# Autodesk Inventor assembly: WedgeBotV3.1
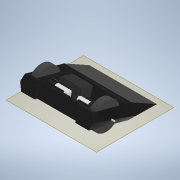
[picture p0: Inventor's stored thumbnail of the model, 180x180]
Saved by Autodesk Inventor 2020 (Build 240168000, 168)
## iProperties
Created: 2023-12-06
Part Number: WedgeBotV3.1
Document SubType Name: Assembly
Designer: smz3rm
Mass: 461.451 g
Surface Area: 1134.27 cm^2
Volume: 369.635 cm^3
Density: 1.2484 g/cm^3
Author: smz3rm
## Documents named in this file (8)
- C:\Users\smz3rm\OneDrive - BP\Documents\DigitalTwin\Models\BattleBot\WedgeBotV3.1.iam
- C:\Users\smz3rm\OneDrive - BP\Documents\DigitalTwin\Models\BattleBot\BodyWedgeWedgeV3.1.ipt
- C:\Users\smz3rm\OneDrive - BP\Documents\DigitalTwin\Models\BattleBot\BodyWedgeBaseV3.1.ipt
- C:\Users\smz3rm\OneDrive - BP\Documents\DigitalTwin\Models\BattleBot\DriveMotorV2.ipt
- C:\Users\smz3rm\OneDrive - BP\Documents\DigitalTwin\Models\BattleBot\BodyWedgeSideV3.1.ipt
- C:\Users\smz3rm\OneDrive - BP\Documents\DigitalTwin\Models\BattleBot\WheelV1.ipt
- C:\Users\smz3rm\OneDrive - BP\Documents\DigitalTwin\Models\BattleBot\HubV2.ipt
- C:\Users\smz3rm\OneDrive - BP\Documents\DigitalTwin\Models\BattleBot\BatteryV1.ipt
## Components (11 placed, 7 different names)
1. BodyWedgeWedgeV3.1:1 — Mate:1, Mate:2, Mate:3, Mate:9, Mate:12, Mate:23
2. BodyWedgeBaseV3.1:1 — Mate:1, Mate:2, Mate:3, Mate:4, Mate:5, Mate:6, Mate:7, Mate:8, Mate:10, Mate:11, Mate:13, Mate:14, Mate:20, Mate:22, Mate:24, Mate:25, Mate:26
3. DriveMotorV2:1 — Mate:7, Mate:8, Mate:19
4. DriveMotorV2:2 — Mate:4, Mate:5, Mate:6, Mate:21
5. BodyWedgeSideV3.1:1 — Mate:12, Mate:13, Mate:14
6. BodyWedgeSideV3.1:2 — Mate:9, Mate:10, Mate:11
7. WheelV1:1 — Mate:15, Mate:16
8. HubV2:1 — Mate:15, Mate:16, Mate:19, Mate:20
9. WheelV1:2 — Mate:17, Mate:18, Tangent:1
10. HubV2:2 — Mate:17, Mate:18, Mate:21, Mate:22
11. BatteryV1:1 — Mate:24, Mate:25, Mate:26
## Relationships (27: Mate 26, Tangent 1)
- Mate:1: BodyWedgeWedgeV3.1:1 ↔ BodyWedgeBaseV3.1:1
- Mate:2: BodyWedgeWedgeV3.1:1 ↔ BodyWedgeBaseV3.1:1
- Mate:3: BodyWedgeWedgeV3.1:1 ↔ BodyWedgeBaseV3.1:1
- Mate:4: BodyWedgeBaseV3.1:1 ↔ DriveMotorV2:2
- Mate:5: BodyWedgeBaseV3.1:1 ↔ DriveMotorV2:2
- Mate:6: BodyWedgeBaseV3.1:1 ↔ DriveMotorV2:2
- Mate:7: BodyWedgeBaseV3.1:1 ↔ DriveMotorV2:1
- Mate:8: BodyWedgeBaseV3.1:1 ↔ DriveMotorV2:1
- Mate:9: BodyWedgeWedgeV3.1:1 ↔ BodyWedgeSideV3.1:2
- Mate:10: BodyWedgeBaseV3.1:1 ↔ BodyWedgeSideV3.1:2
- Mate:11: BodyWedgeBaseV3.1:1 ↔ BodyWedgeSideV3.1:2
- Mate:12: BodyWedgeWedgeV3.1:1 ↔ BodyWedgeSideV3.1:1
- Mate:13: BodyWedgeBaseV3.1:1 ↔ BodyWedgeSideV3.1:1
- Mate:14: BodyWedgeBaseV3.1:1 ↔ BodyWedgeSideV3.1:1
- Mate:15: WheelV1:1 ↔ HubV2:1
- Mate:16: WheelV1:1 ↔ HubV2:1
- Mate:17: WheelV1:2 ↔ HubV2:2
- Mate:18: WheelV1:2 ↔ HubV2:2
- Mate:19: DriveMotorV2:1 ↔ HubV2:1
- Mate:20: BodyWedgeBaseV3.1:1 ↔ HubV2:1
- Mate:21: DriveMotorV2:2 ↔ HubV2:2
- Mate:22: BodyWedgeBaseV3.1:1 ↔ HubV2:2
- Tangent:1: WheelV1:2
- Mate:23: BodyWedgeWedgeV3.1:1
- Mate:24: BodyWedgeBaseV3.1:1 ↔ BatteryV1:1
- Mate:25: BodyWedgeBaseV3.1:1 ↔ BatteryV1:1
- Mate:26: BodyWedgeBaseV3.1:1 ↔ BatteryV1:1
